# Autodesk Inventor assembly: Unidade_de_potência
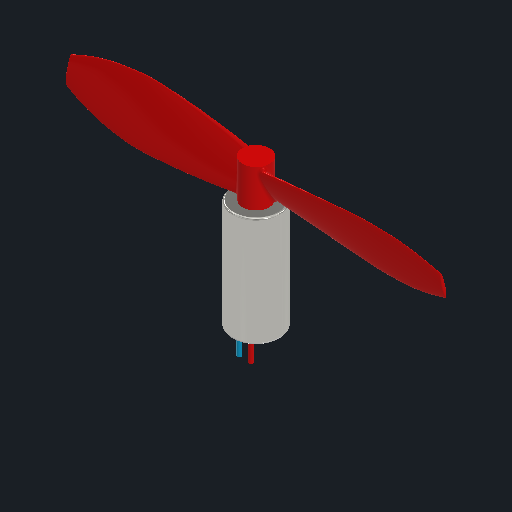
[picture p0: Inventor's stored thumbnail of the model, 512x512]
Saved by Autodesk Inventor 2027 (Build 310192000, 192)
## iProperties
Created: 2026-07-17
Part Number: Unidade_de_potência
Document SubType Name: Assembly
Designer: marcu
Author: marcu
## Documents named in this file (3)
- C:\Users\marcu\projetos\cin-maker\Projeto_drone\Unidade_de_potência.iam
- C:\Users\marcu\projetos\cin-maker\Projeto_drone\Motor.ipt
- C:\Users\marcu\projetos\cin-maker\Projeto_drone\Hélice1.ipt
## Components (2 placed, 2 different names)
1. Motor:1 — Coincidente:1, Coincidente:2
2. Hélice1:1 — Coincidente:1, Coincidente:2
## Relationships (2: Mate 2)
- Coincidente:1 [Mate]: Motor:1 ↔ Hélice1:1
- Coincidente:2 [Mate]: Motor:1 ↔ Hélice1:1
## Named parameters: Finish1_Area = 3.93328, Finish1_Thickness = 0.008 mm, Finish2_Area = 0.0942478, Finish2_Thickness = 0.008 mm, Finish3_Area = 0.0970752, Finish3_Thickness = 0.008 mm, Finish4_Area = 0.0970752, Finish4_Thickness = 0.008 mm
note: some values were not read from the file. Shown as the stored number, unit unknown: "Finish1_Area", "Finish2_Area", "Finish3_Area", "Finish4_Area".
